# Autodesk Inventor assembly: Lamp
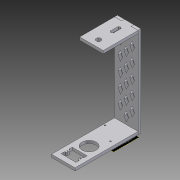
[picture p0: Inventor's stored thumbnail of the model, 180x180]
Saved by Autodesk Inventor 2012 SP2 (Build 160219200, 219)
## iProperties
Created: 2013-03-12
Part Number: Lamp
Document SubType Name: Assembly
Designer: blacki
Author: blacki
## Documents named in this file (5)
- E:\PROJEKTE\WELTHERRSCHAFT\04_SENSELAMP\FRAME\RECTANGULARFRAME\Lamp.iam
- E:\PROJEKTE\WELTHERRSCHAFT\04_SENSELAMP\FRAME\RECTANGULARFRAME\Top.ipt
- E:\PROJEKTE\WELTHERRSCHAFT\04_SENSELAMP\FRAME\RECTANGULARFRAME\Back.ipt
- E:\Projekte\Weltherrschaft\04_SenseLamp\frame\RectangularFrame\Bottom.ipt
- E:\Projekte\Weltherrschaft\04_SenseLamp\frame\RectangularFrame\TLwr703n_image.ipt
## Components (4 placed, 4 different names)
1. Top:1 — Flush:2, Mate:1, Mate:2
2. Back:1 — Flush:2, Mate:1, Mate:2, Flush:3, Flush:4, Flush:5
3. BOTTOM:1 — Flush:3, Flush:4, Flush:5, Mate:3, Flush:6
4. TLwr703n_image:1 — Mate:3, Flush:6
## Relationships (8: Flush 5, Mate 3)
- Flush:2: Top:1 ↔ Back:1
- Mate:1: Top:1 ↔ Back:1
- Mate:2: Top:1 ↔ Back:1
- Flush:3: Back:1 ↔ BOTTOM:1
- Flush:4: Back:1 ↔ BOTTOM:1
- Flush:5: Back:1 ↔ BOTTOM:1
- Mate:3: BOTTOM:1 ↔ TLwr703n_image:1
- Flush:6 (10 mm): BOTTOM:1 ↔ TLwr703n_image:1
